# Autodesk Inventor assembly: Chuck with Tamale Assembly Plate
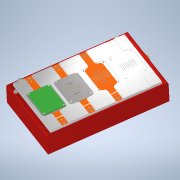
[picture p0: Inventor's stored thumbnail of the model, 180x180]
Saved by Autodesk Inventor 2022 (Build 260153000, 153)
## iProperties
Created: 2021-07-20
Part Number: Chuck with Tamale Assembly Plate
Document SubType Name: Assembly
Designer: Caleb
Author: Caleb
## Documents named in this file (3)
- C:\Users\Caleb\Desktop\nebraska-silicon-lab\Hardware\ETL\Module Assembly\Chuck with Tamale Assembly Plate.iam
- C:\Users\Caleb\Desktop\nebraska-silicon-lab\Hardware\ETL\Module Assembly\Chuck - V2\Chuck - V2.iam
- C:\Users\Caleb\Desktop\nebraska-silicon-lab\Hardware\ETL\Module Assembly\Tamale Assembly Plate\Plate Assembly.iam
## Components (2 placed, 2 different names)
1. Chuck - V2:1 [sub-assembly] — Mate:1, Angle:1, Tangent:1, Tangent:2
2. Plate Assembly:1 [sub-assembly] — Mate:1, Angle:1, Tangent:1, Tangent:2
## Relationships (4: Tangent 2, Mate 1, Angle 1)
- Mate:1: Chuck - V2:1 ↔ Plate Assembly:1
- Angle:1 (0 deg): Chuck - V2:1 ↔ Plate Assembly:1
- Tangent:1: Chuck - V2:1 ↔ Plate Assembly:1
- Tangent:2: Chuck - V2:1 ↔ Plate Assembly:1
